# Autodesk Inventor assembly: main assembly
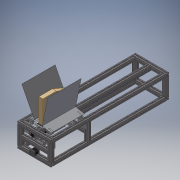
[picture p0: Inventor's stored thumbnail of the model, 180x180]
Saved by Autodesk Inventor 2016 SP1 (Build 200210100, 210)
## iProperties
Created: 2016-05-25
Part Number: main assembly
Document SubType Name: Assembly
Designer: ubik
Author: ubik
## Documents named in this file (24)
- E:\GitHub\glue-filter\hardware\inventor\main assembly.iam
- E:\GitHub\glue-filter\hardware\inventor\30x30\30x30-01.ipt
- E:\GitHub\glue-filter\hardware\inventor\30x30.ipt
- E:\GitHub\glue-filter\hardware\inventor\mobile bottom plate.ipt
- E:\GitHub\glue-filter\hardware\inventor\mobile vertical plate.ipt
- E:\GitHub\glue-filter\hardware\inventor\mobile top plate.ipt
- E:\GitHub\glue-filter\hardware\inventor\filter base.ipt
- E:\GitHub\glue-filter\hardware\inventor\filter top plate.ipt
- E:\GitHub\glue-filter\hardware\inventor\filter top.ipt
- E:\GitHub\glue-filter\hardware\inventor\gear.ipt
- E:\GitHub\glue-filter\hardware\inventor\bearing support.ipt
- E:\GitHub\glue-filter\hardware\inventor\sheet support.ipt
- E:\GitHub\glue-filter\hardware\inventor\NEMA17 Stepper.ipt
- E:\GitHub\glue-filter\hardware\inventor\nema17 x plate.ipt
- E:\GitHub\glue-filter\hardware\inventor\30x30\30x30-02.ipt
- E:\GitHub\glue-filter\hardware\inventor\30x30\30x30-03.ipt
- E:\GitHub\glue-filter\hardware\inventor\30x30\30x30-04.ipt
- E:\GitHub\glue-filter\hardware\inventor\HSR20-xxxx\HSR20-xxxx-01.ipt
- E:\GitHub\glue-filter\hardware\inventor\HSR20-xxxx.ipt
- E:\GitHub\glue-filter\hardware\inventor\HSR20.ipt
- E:\GitHub\glue-filter\hardware\inventor\gear guide.ipt
- E:\GitHub\glue-filter\hardware\inventor\top guide support plate.ipt
- E:\GitHub\glue-filter\hardware\inventor\5mm guide.ipt
- E:\GitHub\glue-filter\hardware\inventor\chuck support.ipt
## Components (46 placed, 21 different names)
1. 30x30-01:1 — Mate:26, Flush:24, Flush:25, Mate:27, Flush:26, Flush:27, Flush:29, Mate:28, Mate:43, Flush:63
2. mobile bottom plate:1 — Mate:7, Flush:7, Flush:8, Mate:8, Flush:9, Flush:10, Mate:42, Mate:47, Flush:64
3. mobile vertical plate:1 — Mate:7, Flush:7, Flush:9, Flush:12, Mate:9
4. mobile vertical plate:2 — Flush:8, Mate:8, Flush:10, Flush:11, Mate:48
5. mobile top plate:1 — Flush:11, Flush:12, Mate:9, Mate:10, Flush:13, Flush:14
6. filter base:1 — Mate:11, Mate:12, Mate:13, Mate:14, Flush:15, Flush:16
7. filter top plate:1 — Mate:10, Flush:13, Flush:14, Mate:11, Mate:12, Mate:13, Flush:21
8. filter top:1 — Mate:14, Flush:15, Flush:16
9. gear:1 — Tangent:3, Flush:17, Mate:52, Mate:56
10. gear:2 — Tangent:3, Flush:17, Mate:50, Mate:51
11. bearing support:1 — Mate:49, Mate:50, Mate:51, Mate:52, Flush:65, Mate:53, Mate:54
12. sheet support:1 — Flush:22, Mate:72, Flush:81, Flush:82, Flush:83
13. sheet support:2 — Flush:21, Flush:22, Mate:71, Mate:73, Flush:78, Flush:79, Flush:80
14. NEMA17 Stepper:1 — Flush:23, Mate:24, Mate:25
15. nema17 x plate:1 — Flush:23, Mate:24, Mate:25, Mate:26, Flush:24, Flush:25
16. 30x30-02:3 — Mate:27, Flush:26, Flush:28, Flush:29, Mate:29, Flush:30, Flush:31, Flush:33, Flush:49, Flush:50, Mate:33, Mate:35, Flush:54, Mate:44
17. 30x30-02:4 — Flush:27, Flush:28, Mate:28, Flush:38, Flush:39, Mate:30, Mate:31, Flush:40
18. 30x30-03:5 — Flush:32, Flush:33, Flush:34, Flush:41, Flush:42, Mate:32, Mate:34, Mate:39, Mate:40, Flush:60, Mate:53, Mate:61
19. 30x30-03:6 — Mate:29, Flush:30, Flush:31, Flush:32, Flush:34, Flush:53, Flush:55, Mate:36, Flush:72
20. 30x30-03:7 — Flush:36, Flush:37, Flush:39, Mate:30, Flush:47, Flush:48
21. 30x30-03:8 — Flush:36, Flush:37, Flush:38, Mate:31, Flush:40
22. 30x30-02:9 — Flush:41, Flush:42, Mate:32, Flush:46, Flush:52, Flush:56
23. 30x30-02:10 — Flush:46, Flush:47, Flush:48
24. 30x30-01:12 — Mate:35, Flush:53, Flush:54, Mate:66
25. 30x30-01:13 — Flush:49, Flush:50, Mate:33, Flush:51, Mate:63
26. 30x30-01:14 — Flush:51, Mate:34, Flush:52, Mate:37, Flush:57
27. 30x30-01:15 — Flush:55, Mate:36, Flush:56, Mate:38, Flush:58
28. 30x30-03:16 — Mate:38, Flush:58, Flush:59, Flush:61, Mate:65
29. 30x30-03:17 — Mate:37, Flush:57, Mate:39, Flush:59, Mate:41, Flush:67, Mate:60
30. 30x30-04:18 — Mate:40, Flush:60, Flush:62, Mate:42, Mate:49, Flush:65
31. 30x30-04:19 — Mate:41, Flush:61, Flush:62, Mate:55, Flush:66, Mate:58, Flush:84
32. HSR20-xxxx-01:2 — Mate:43, Mate:44, Flush:63, Mate:45, Mate:46
33. HSR20:1 — Mate:45, Mate:46, Mate:47, Flush:64, Mate:48
34. NEMA17 Stepper:2 — Mate:54
35. bearing support:2 — Mate:55, Flush:66, Mate:56, Mate:57, Flush:84
36. gear guide:1 — Mate:57, Mate:58
37. top guide support plate:1 — Flush:71, Flush:72, Mate:64, Flush:73, Flush:74, Flush:75, Mate:66, Mate:73
38. top guide support plate:2 — Flush:67, Flush:68, Flush:69, Mate:60, Mate:63
39. top guide support plate:3 — Flush:68, Flush:69, Mate:61, Mate:62, Flush:70, Flush:71
40. top guide support plate:4 — Flush:74, Flush:75, Mate:65
41. 5mm guide:1 — Mate:62, Flush:70, Mate:67, Mate:68
42. 5mm guide:2 — Mate:64, Flush:73, Mate:69, Mate:70
43. chuck support:1 — Mate:67, Flush:76, Mate:72, Flush:81
44. chuck support:2 — Mate:68, Flush:76, Flush:82, Flush:83
45. chuck support:3 — Mate:70, Flush:77, Flush:78, Flush:80
46. chuck support:4 — Mate:69, Flush:77, Mate:71, Flush:79
## Relationships (129: Flush 71, Mate 57, Tangent 1)
- Mate:7: mobile bottom plate:1 ↔ mobile vertical plate:1
- Flush:7: mobile bottom plate:1 ↔ mobile vertical plate:1
- Flush:8: mobile bottom plate:1 ↔ mobile vertical plate:2
- Mate:8: mobile bottom plate:1 ↔ mobile vertical plate:2
- Flush:9: mobile bottom plate:1 ↔ mobile vertical plate:1
- Flush:10: mobile bottom plate:1 ↔ mobile vertical plate:2
- Flush:11: mobile vertical plate:2 ↔ mobile top plate:1
- Flush:12 (-2 mm): mobile vertical plate:1 ↔ mobile top plate:1
- Mate:9: mobile vertical plate:1 ↔ mobile top plate:1
- Mate:10: mobile top plate:1 ↔ filter top plate:1
- Flush:13 (50 mm): mobile top plate:1 ↔ filter top plate:1
- Flush:14 (2 mm): mobile top plate:1 ↔ filter top plate:1
- Mate:11: filter base:1 ↔ filter top plate:1
- Mate:12: filter base:1 ↔ filter top plate:1
- Mate:13: filter base:1 ↔ filter top plate:1
- Mate:14: filter base:1 ↔ filter top:1
- Flush:15 (-11 mm): filter base:1 ↔ filter top:1
- Flush:16 (10 mm): filter base:1 ↔ filter top:1
- Tangent:3: gear:1 ↔ gear:2
- Flush:17: gear:1 ↔ gear:2
- Flush:21: filter top plate:1 ↔ sheet support:2
- Flush:22: sheet support:1 ↔ sheet support:2
- Flush:23: NEMA17 Stepper:1 ↔ nema17 x plate:1
- Mate:24: NEMA17 Stepper:1 ↔ nema17 x plate:1
- Mate:25: NEMA17 Stepper:1 ↔ nema17 x plate:1
- Mate:26: 30x30-01:1 ↔ nema17 x plate:1
- Flush:24: 30x30-01:1 ↔ nema17 x plate:1
- Flush:25: 30x30-01:1 ↔ nema17 x plate:1
- Mate:27: 30x30-01:1 ↔ 30x30-02:3
- Flush:26: 30x30-01:1 ↔ 30x30-02:3
- Flush:27: 30x30-01:1 ↔ 30x30-02:4
- Flush:28: 30x30-02:3 ↔ 30x30-02:4
- Flush:29 (135 mm): 30x30-01:1 ↔ 30x30-02:3
- Mate:28: 30x30-01:1 ↔ 30x30-02:4
- Mate:29: 30x30-02:3 ↔ 30x30-03:6
- Flush:30: 30x30-02:3 ↔ 30x30-03:6
- Flush:31: 30x30-02:3 ↔ 30x30-03:6
- Flush:32: 30x30-03:5 ↔ 30x30-03:6
- Flush:33: 30x30-02:3 ↔ 30x30-03:5
- Flush:34: 30x30-03:5 ↔ 30x30-03:6
- Flush:36: 30x30-03:7 ↔ 30x30-03:8
- Flush:37: 30x30-03:7 ↔ 30x30-03:8
- Flush:38: 30x30-02:4 ↔ 30x30-03:8
- Flush:39: 30x30-02:4 ↔ 30x30-03:7
- Mate:30: 30x30-02:4 ↔ 30x30-03:7
- Mate:31: 30x30-02:4 ↔ 30x30-03:8
- Flush:40: 30x30-02:4 ↔ 30x30-03:8
- Flush:41: 30x30-03:5 ↔ 30x30-02:9
- Flush:42: 30x30-03:5 ↔ 30x30-02:9
- Mate:32: 30x30-03:5 ↔ 30x30-02:9
- Flush:46: 30x30-02:9 ↔ 30x30-02:10
- Flush:47: 30x30-03:7 ↔ 30x30-02:10
- Flush:48: 30x30-03:7 ↔ 30x30-02:10
- Flush:49: 30x30-02:3 ↔ 30x30-01:13
- Flush:50: 30x30-02:3 ↔ 30x30-01:13
- Mate:33: 30x30-02:3 ↔ 30x30-01:13
- Flush:51: 30x30-01:13 ↔ 30x30-01:14
- Mate:34: 30x30-03:5 ↔ 30x30-01:14
- Flush:52: 30x30-02:9 ↔ 30x30-01:14
- Mate:35: 30x30-02:3 ↔ 30x30-01:12
- Flush:53: 30x30-03:6 ↔ 30x30-01:12
- Flush:54: 30x30-02:3 ↔ 30x30-01:12
- Flush:55: 30x30-03:6 ↔ 30x30-01:15
- Mate:36: 30x30-03:6 ↔ 30x30-01:15
- Flush:56: 30x30-02:9 ↔ 30x30-01:15
- Mate:37: 30x30-01:14 ↔ 30x30-03:17
- Flush:57: 30x30-01:14 ↔ 30x30-03:17
- Mate:38: 30x30-01:15 ↔ 30x30-03:16
- Flush:58: 30x30-01:15 ↔ 30x30-03:16
- Mate:39 (300 mm): 30x30-03:5 ↔ 30x30-03:17
- Flush:59: 30x30-03:16 ↔ 30x30-03:17
- Mate:40: 30x30-03:5 ↔ 30x30-04:18
- Flush:60: 30x30-03:5 ↔ 30x30-04:18
- Mate:41: 30x30-03:17 ↔ 30x30-04:19
- Flush:61: 30x30-03:16 ↔ 30x30-04:19
- Flush:62: 30x30-04:18 ↔ 30x30-04:19
- Mate:42 (25 mm): mobile bottom plate:1 ↔ 30x30-04:18
- Mate:43: 30x30-01:1 ↔ HSR20-xxxx-01:2
- Mate:44: 30x30-02:3 ↔ HSR20-xxxx-01:2
- Flush:63 (5 mm): 30x30-01:1 ↔ HSR20-xxxx-01:2
- Mate:45 (1 mm): HSR20-xxxx-01:2 ↔ HSR20:1
- Mate:46: HSR20-xxxx-01:2 ↔ HSR20:1
- Mate:47: mobile bottom plate:1 ↔ HSR20:1
- Flush:64: mobile bottom plate:1 ↔ HSR20:1
- Mate:48 (2 mm): mobile vertical plate:2 ↔ HSR20:1
- Mate:49: bearing support:1 ↔ 30x30-04:18
- Mate:50 (20 mm): gear:2 ↔ bearing support:1
- Mate:51: gear:2 ↔ bearing support:1
- Mate:52: gear:1 ↔ bearing support:1
- Flush:65: bearing support:1 ↔ 30x30-04:18
- Mate:53 (75 mm): bearing support:1 ↔ 30x30-03:5
- Mate:54: bearing support:1 ↔ NEMA17 Stepper:2
- Mate:55: 30x30-04:19 ↔ bearing support:2
- Flush:66: 30x30-04:19 ↔ bearing support:2
- Mate:56: gear:1 ↔ bearing support:2
- Mate:57: bearing support:2 ↔ gear guide:1
- Mate:58: 30x30-04:19 ↔ gear guide:1
- Flush:67: 30x30-03:17 ↔ top guide support plate:2
- Flush:68: top guide support plate:2 ↔ top guide support plate:3
- Flush:69: top guide support plate:2 ↔ top guide support plate:3
- Mate:60: 30x30-03:17 ↔ top guide support plate:2
- Mate:61: 30x30-03:5 ↔ top guide support plate:3
- Mate:62: top guide support plate:3 ↔ 5mm guide:1
- Flush:70: top guide support plate:3 ↔ 5mm guide:1
- Mate:63: 30x30-01:13 ↔ top guide support plate:2
- Flush:71: top guide support plate:1 ↔ top guide support plate:3
- Flush:72: 30x30-03:6 ↔ top guide support plate:1
- Mate:64: top guide support plate:1 ↔ 5mm guide:2
- Flush:73: top guide support plate:1 ↔ 5mm guide:2
- Flush:74: top guide support plate:1 ↔ top guide support plate:4
- Flush:75: top guide support plate:1 ↔ top guide support plate:4
- Mate:65: 30x30-03:16 ↔ top guide support plate:4
- Mate:66: 30x30-01:12 ↔ top guide support plate:1
- Mate:67: 5mm guide:1 ↔ chuck support:1
- Mate:68: 5mm guide:1 ↔ chuck support:2
- Flush:76: chuck support:1 ↔ chuck support:2
- Mate:69: 5mm guide:2 ↔ chuck support:4
- Mate:70: 5mm guide:2 ↔ chuck support:3
- Flush:77: chuck support:3 ↔ chuck support:4
- Mate:71: sheet support:2 ↔ chuck support:4
- Mate:72: sheet support:1 ↔ chuck support:1
- Mate:73 (5 mm): sheet support:2 ↔ top guide support plate:1
- Flush:78: sheet support:2 ↔ chuck support:3
- Flush:79 (15 mm): sheet support:2 ↔ chuck support:4
- Flush:80 (15 mm): sheet support:2 ↔ chuck support:3
- Flush:81 (15 mm): sheet support:1 ↔ chuck support:1
- Flush:82 (15 mm): sheet support:1 ↔ chuck support:2
- Flush:83: sheet support:1 ↔ chuck support:2
- Flush:84: 30x30-04:19 ↔ bearing support:2
